# Autodesk Inventor assembly: SCST10-8
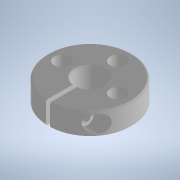
[picture p0: Inventor's stored thumbnail of the model, 180x180]
Saved by Autodesk Inventor 2021 (Build 250183000, 183)
## iProperties
Category: PARTsolutions
Company: MISUMI
Created: 2025-09-06
Part Number: SCST10-8
Catalog Web Link: www.cadenas.de
Description: SCST, PSCST, SSCST, SCSTR, PSCSTR, SSCSTR-Set Collars - Slit 3 Hole/3 Tap - Standard Type -
Vendor: MISUMI
Document SubType Name: Assembly
Designer: psAdmin
Manufacturer: MISUMI
Mass: 4.17999 g
Surface Area: 30.2634 cm^2
Volume: 4.17999 cm^3
Density: 1 g/cm^3
Title: SCST10-8
Author: Cadenas PARTsolutions
Comments: Set Collars - Slit 3 Hole/3 Tap - Standard Type -
PSOL_IDENT_0: {$CADENAS_DATA/23d-libs/misumi/metric/03_set_collars/scst_asmtab.prj},219 {VTYP=3D},{STYP=ASSTAB},{N
PSOL_IDENT_1: B=SCST10-8},{LINA=SCST10-8},{NN=SCST, PSCST, SSCST, SCSTR, PSCSTR, SSCSTR},{DATE=29.11.2024 04:05:21
PSOL_IDENT_2: },{GEOMDATE=15.09.2021 06:07:55},{VERSION=},{LINEID=60},{WBVAR=TS,MAT,ST,BS},{WBNUMERIC=BS}  {NB=SCS
PSOL_IDENT_3: T10-8},{LINA=SCST10-8},{KT=DUMMY},{PN=SCST10-8},{TYPE=SCST},{TS=3H},{TSALG= '3H' , '3-Hole' , '3T' ,
PSOL_IDENT_4: '3-Tapped' },{MAT=S45C},{ST=BO},{STALG= 'BO' , 'Black Oxide' , 'ENP' , 'Electroless Nickel Plating'
PSOL_IDENT_5: },{AC=Hex Socket Head Cap Screw 1 pc.},{ACMAT=4137 Alloy Steel},{D=10},{BS=8},{BALG= 8 , 10 , 12 ,1
PSOL_IDENT_6: 5 },{D1=30},{M=M3},{M3D=3},{DD=3.4},{R=3.00},{W=1.5},{X=9.0},{Y=5},{P=20},{C=0.5},{S=5.5},{M1=-},{M1
PSOL_IDENT_7: 3D=0},{L=14},{PPATH=scst/scst_templ.prj}
NB: SCST10-8
NN: SCST, PSCST, SSCST, SCSTR, PSCSTR, SSCSTR
NT: Set Collars - Slit 3 Hole/3 Tap - Standard Type -
NBSYN: $PN.
LINA: SCST10-8
CATALOG: Misumi
PN: SCST10-8
TS: 3-Hole
MAT: 1045 Carbon Steel
ST: Black Oxide
AC: Hex Socket Head Cap Screw 1 pc.
ACMAT: 4137 Alloy Steel
D: 10
BS: 8
D1: 30
M: M3
DD: 3.4
R: 3
W: 1.5
X: 9
Y: 5
P: 20
C: 0.5
S: 5.5
M1: -
SUPPLIER: MISUMI
ARTICLENO: SCST10-8
BOMINFO: SCST10-8
CREATOR: CADENAS GmbH
## Documents named in this file (3)
- e:\temp\worker_COMMON_114\temp\tmp_2956_346_TMZsF\format_0\SCST10-8.iam
- e:\temp\worker_COMMON_114\temp\tmp_2956_346_TMZsF\format_0\SCST10-8b.ipt
- e:\temp\worker_COMMON_114\temp\tmp_2956_346_TMZsF\format_0\BOLT3-14.ipt
## Components (2 placed, 2 different names)
1. SCST10-8b:1 — to_bolt_XY@1 <-> to_cp_XY@2, to_bolt_Z@1 <-> to_cp_Z@2, to_bolt_YZ@1 <-> to_cp_YZ@2
2. BOLT3-14:1 — to_bolt_XY@1 <-> to_cp_XY@2, to_bolt_Z@1 <-> to_cp_Z@2, to_bolt_YZ@1 <-> to_cp_YZ@2
## Relationships (3: Mate 2, Angle 1)
- to_bolt_XY@1 <-> to_cp_XY@2 [Mate]: SCST10-8b:1 ↔ BOLT3-14:1
- to_bolt_Z@1 <-> to_cp_Z@2 [Mate]: SCST10-8b:1 ↔ BOLT3-14:1
- to_bolt_YZ@1 <-> to_cp_YZ@2 [Angle] (0 deg): SCST10-8b:1 ↔ BOLT3-14:1
